# Autodesk Inventor assembly: intake1.0
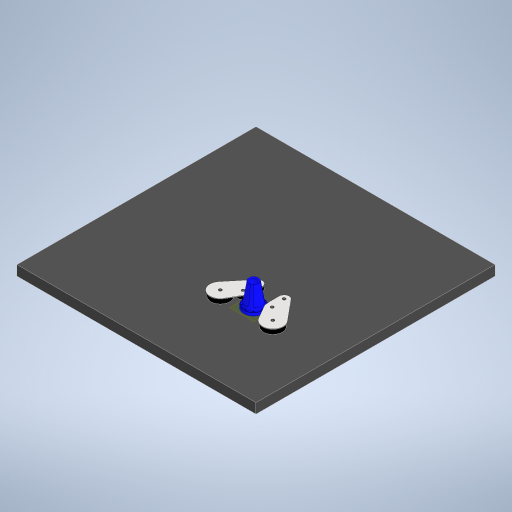
[picture p0: Inventor's stored thumbnail of the model, 512x512]
Saved by Autodesk Inventor 2023 (Build 270158000, 158)
## iProperties
Created: 2022-09-11
Part Number: intake1.0
Document SubType Name: Assembly
Designer: deli
Author: deli
## Documents named in this file (12)
- C:\Users\deli\OneDrive - Eastside Preparatory School\FTC\8103-power-play\CAD\intake1.0.iam
- C:\Users\deli\OneDrive - Eastside Preparatory School\FTC\8103-power-play\CAD\FTC-parts\am-4801_Blue am-4801_Red Cone REV2.ipt
- C:\Users\deli\OneDrive - Eastside Preparatory School\FTC\8103-power-play\CAD\Field Mat.ipt
- C:\Users\deli\OneDrive - Eastside Preparatory School\FTC\8103-power-play\CAD\IntakeHolder.ipt
- C:\Users\deli\OneDrive - Eastside Preparatory School\FTC\8103-power-play\CAD\FTC-parts\goBILDA\1611-0514-4008.ipt
- C:\Users\deli\OneDrive - Eastside Preparatory School\FTC\8103-power-play\CAD\FTC-parts\goBILDA\3613-4008-0048.ipt
- C:\Users\deli\OneDrive - Eastside Preparatory School\FTC\8103-power-play\CAD\FTC-parts\goBILDA\2801-0004-0011.ipt
- C:\Users\deli\OneDrive - Eastside Preparatory School\FTC\8103-power-play\CAD\FTC-parts\goBILDA\2802-0004-0010.ipt
- C:\Users\deli\OneDrive - Eastside Preparatory School\FTC\8103-power-play\CAD\FTC-parts\goBILDA\3613-0014-0096.ipt
- C:\Users\deli\OneDrive - Eastside Preparatory School\FTC\8103-power-play\CAD\FTC-parts\goBILDA\1309-0016-4008 assembly.ipt
- C:\Users\deli\OneDrive - Eastside Preparatory School\FTC\8103-power-play\CAD\FTC-parts\goBILDA\1522-0010-0020.ipt
- C:\Users\deli\OneDrive - Eastside Preparatory School\FTC\8103-power-play\CAD\FTC-parts\goBILDA\1522-0010-0040.ipt
## Components (31 placed, 11 different names)
1. am-4801_Blue am-4801_Red Cone REV2:1 — Mate:1
2. Field Mat:1 — Mate:1, Mate:79, Angle:1
3. IntakeHolder:1 — Mate:2, Mate:3, Mate:4, Mate:5, Mate:6, Mate:7, Mate:8, Mate:9, Mate:43, Mate:44, Mate:45, Mate:46, Angle:1
4. 1611-0514-4008:1 — Mate:2, Mate:8, Mate:66, Mate:67
5. 1611-0514-4008:2 — Mate:5, Mate:6, Mate:62, Mate:63
6. 1611-0514-4008:3 — Mate:4, Mate:7, Mate:64, Mate:65
7. 1611-0514-4008:4 — Mate:3, Mate:9, Mate:70, Mate:71
8. 3613-4008-0048:1 — Mate:26, Mate:27, Mate:56, Mate:57
9. 3613-4008-0048:2 — Mate:28, Mate:29, Mate:54, Mate:55, Mate:71
10. 3613-4008-0048:3 — Mate:32, Mate:33, Mate:60, Mate:61
11. 3613-4008-0048:4 — Mate:30, Mate:31, Mate:58, Mate:59, Mate:63
12. 2801-0004-0011:1 — Mate:32, Mate:33, Mate:40, Mate:41
13. 2801-0004-0011:2 — Mate:26, Mate:27, Mate:68, Mate:69
14. 2801-0004-0011:3 — Mate:28, Mate:29, Mate:36, Mate:37
15. 2801-0004-0011:4 — Mate:30, Mate:31, Mate:38, Mate:39
16. 2802-0004-0010:5 — Mate:38, Mate:39
17. 2802-0004-0010:6 — Mate:40, Mate:41
18. 2802-0004-0010:7 — Mate:36, Mate:37
19. 2802-0004-0010:8 — Mate:68, Mate:69
20. 1611-0514-4008:5 — Mate:43, Mate:44, Mate:52, Mate:53
21. 1611-0514-4008:6 — Mate:45, Mate:46, Mate:77, Mate:78
22. 3613-0014-0096:1 — Mate:47, Mate:48, Mate:49, Mate:79
23. 1309-0016-4008 assembly:1 — Mate:47, Mate:48, Mate:49, Mate:50, Mate:51
24. 1522-0010-0020:1 — Mate:50, Mate:51, Mate:52, Mate:53
25. 1522-0010-0040:1 — Mate:54, Mate:55, Mate:70
26. 1522-0010-0040:2 — Mate:56, Mate:57, Mate:66, Mate:67
27. 1522-0010-0040:3 — Mate:58, Mate:59, Mate:62
28. 1522-0010-0040:4 — Mate:60, Mate:61, Mate:64, Mate:65
29. 3613-0014-0096:2 — Mate:78
30. 1309-0016-4008 assembly:2
31. 1522-0010-0020:2 — Mate:77
## Relationships (61: Mate 60, Angle 1)
- Mate:1 (5.461 mm): am-4801_Blue am-4801_Red Cone REV2:1 ↔ Field Mat:1
- Mate:2: IntakeHolder:1 ↔ 1611-0514-4008:1
- Mate:3: IntakeHolder:1 ↔ 1611-0514-4008:4
- Mate:4: IntakeHolder:1 ↔ 1611-0514-4008:3
- Mate:5: IntakeHolder:1 ↔ 1611-0514-4008:2
- Mate:6: IntakeHolder:1 ↔ 1611-0514-4008:2
- Mate:7: IntakeHolder:1 ↔ 1611-0514-4008:3
- Mate:8: IntakeHolder:1 ↔ 1611-0514-4008:1
- Mate:9: IntakeHolder:1 ↔ 1611-0514-4008:4
- Mate:26: 3613-4008-0048:1 ↔ 2801-0004-0011:2
- Mate:27: 3613-4008-0048:1 ↔ 2801-0004-0011:2
- Mate:28: 3613-4008-0048:2 ↔ 2801-0004-0011:3
- Mate:29: 3613-4008-0048:2 ↔ 2801-0004-0011:3
- Mate:30: 3613-4008-0048:4 ↔ 2801-0004-0011:4
- Mate:31: 3613-4008-0048:4 ↔ 2801-0004-0011:4
- Mate:32: 3613-4008-0048:3 ↔ 2801-0004-0011:1
- Mate:33: 3613-4008-0048:3 ↔ 2801-0004-0011:1
- Mate:36: 2801-0004-0011:3 ↔ 2802-0004-0010:7
- Mate:37: 2801-0004-0011:3 ↔ 2802-0004-0010:7
- Mate:38: 2801-0004-0011:4 ↔ 2802-0004-0010:5
- Mate:39: 2801-0004-0011:4 ↔ 2802-0004-0010:5
- Mate:40: 2801-0004-0011:1 ↔ 2802-0004-0010:6
- Mate:41: 2801-0004-0011:1 ↔ 2802-0004-0010:6
- Mate:43: IntakeHolder:1 ↔ 1611-0514-4008:5
- Mate:44: IntakeHolder:1 ↔ 1611-0514-4008:5
- Mate:45: IntakeHolder:1 ↔ 1611-0514-4008:6
- Mate:46: IntakeHolder:1 ↔ 1611-0514-4008:6
- Mate:47: 3613-0014-0096:1 ↔ 1309-0016-4008 assembly:1
- Mate:48: 3613-0014-0096:1 ↔ 1309-0016-4008 assembly:1
- Mate:49: 3613-0014-0096:1 ↔ 1309-0016-4008 assembly:1
- Mate:50: 1309-0016-4008 assembly:1 ↔ 1522-0010-0020:1
- Mate:51: 1309-0016-4008 assembly:1 ↔ 1522-0010-0020:1
- Mate:52: 1611-0514-4008:5 ↔ 1522-0010-0020:1
- Mate:53: 1611-0514-4008:5 ↔ 1522-0010-0020:1
- Mate:54: 3613-4008-0048:2 ↔ 1522-0010-0040:1
- Mate:55: 3613-4008-0048:2 ↔ 1522-0010-0040:1
- Mate:56: 3613-4008-0048:1 ↔ 1522-0010-0040:2
- Mate:57: 3613-4008-0048:1 ↔ 1522-0010-0040:2
- Mate:58: 3613-4008-0048:4 ↔ 1522-0010-0040:3
- Mate:59: 3613-4008-0048:4 ↔ 1522-0010-0040:3
- Mate:60: 3613-4008-0048:3 ↔ 1522-0010-0040:4
- Mate:61: 3613-4008-0048:3 ↔ 1522-0010-0040:4
- Mate:62: 1611-0514-4008:2 ↔ 1522-0010-0040:3
- Mate:63: 1611-0514-4008:2 ↔ 3613-4008-0048:4
- Mate:64: 1611-0514-4008:3 ↔ 1522-0010-0040:4
- Mate:65: 1611-0514-4008:3 ↔ 1522-0010-0040:4
- Mate:66: 1611-0514-4008:1 ↔ 1522-0010-0040:2
- Mate:67: 1611-0514-4008:1 ↔ 1522-0010-0040:2
- Mate:68: 2801-0004-0011:2 ↔ 2802-0004-0010:8
- Mate:69: 2801-0004-0011:2 ↔ 2802-0004-0010:8
- Mate:70: 1611-0514-4008:4 ↔ 1522-0010-0040:1
- Mate:71: 1611-0514-4008:4 ↔ 3613-4008-0048:2
- [Mate]: 3613-0014-0096:2 ↔ 1309-0016-4008 assembly:2
- [Mate]: 3613-0014-0096:2 ↔ 1309-0016-4008 assembly:2
- [Mate]: 3613-0014-0096:2 ↔ 1309-0016-4008 assembly:2
- [Mate]: 1309-0016-4008 assembly:2 ↔ 1522-0010-0020:2
- [Mate]: 1309-0016-4008 assembly:2 ↔ 1522-0010-0020:2
- Mate:77: 1611-0514-4008:6 ↔ 1522-0010-0020:2
- Mate:78: 1611-0514-4008:6 ↔ 3613-0014-0096:2
- Mate:79 (4 mm): Field Mat:1 ↔ 3613-0014-0096:1
- Angle:1 (5 deg): Field Mat:1 ↔ IntakeHolder:1
## Named parameters: d80_d55 = 0 mm, d81_d56 = 0 mm, d82_d57 = 0 mm, d83_d58 = 0 mm, d84_d59 = 0 mm
